# Autodesk Inventor assembly: hashikadai1
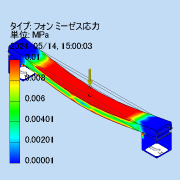
[picture p0: Inventor's stored thumbnail of the model, 180x180]
Saved by Autodesk Inventor 2022 (Build 260153000, 153)
## iProperties
Created: 2024-05-14
Part Number: hashikadai1
Document SubType Name: Assembly
Designer: ktamu
Author: ktamu
## Documents named in this file (9)
- D:\SDinventor\DesignHashi\DesignHashi2-2\hashikadai1.iam
- D:\SDinventor\DesignHashi\DesignHashi2-2\hashgeta1.ipt
- D:\SDinventor\DesignHashi\DesignHashi2-2\hashi1shado.ipt
- D:\SDinventor\DesignHashi\DesignHashi2-2\hashikadai1\AIP\FEA\ep6vs5l7k.fins
- D:\SDinventor\DesignHashi\DesignHashi2-2\hashikadai1\AIP\FEA\ep6vs5l7k.fsat
- D:\SDinventor\DesignHashi\DesignHashi2-2\hashikadai1\AIP\FEA\ep6vs5l7k.ftes
- D:\SDinventor\DesignHashi\DesignHashi2-2\hashikadai1\AIP\FEA\ep6vs5l7k.fwiz
- D:\SDinventor\DesignHashi\DesignHashi2-2\hashikadai1\AIP\FEA\ep6vs5l9c.fmsh
- D:\SDinventor\DesignHashi\DesignHashi2-2\hashikadai1\AIP\FEA\ep6vs5l9d.fres
## Components (3 placed, 2 different names)
1. hashgeta1:1 — フラッシュ:2, フラッシュ:3
2. hashi1shado:1 — フラッシュ:1, フラッシュ:2, フラッシュ:3, フラッシュ:4
3. hashgeta1:2 — フラッシュ:1, フラッシュ:4
## Relationships (4: Flush 4)
- フラッシュ:1 [Flush]: hashi1shado:1 ↔ hashgeta1:2
- フラッシュ:2 [Flush]: hashgeta1:1 ↔ hashi1shado:1
- フラッシュ:3 [Flush]: hashgeta1:1 ↔ hashi1shado:1
- フラッシュ:4 [Flush]: hashi1shado:1 ↔ hashgeta1:2
